# Autodesk Inventor assembly: Assembly1
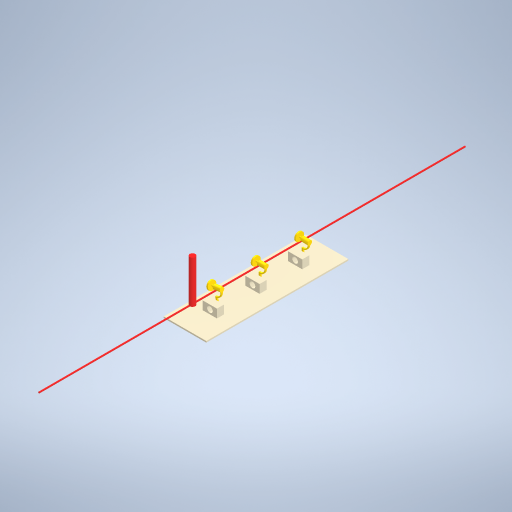
[picture p0: Inventor's stored thumbnail of the model, 512x512]
Saved by Autodesk Inventor 2024 (Build 280153000, 153)
## iProperties
Created: 2024-09-18
Part Number: Assembly1
Document SubType Name: Assembly
Designer: manas
Author: manas
## Documents named in this file (4)
- C:\Users\manas\Downloads\Assembly1.iam
- C:\Users\manas\Downloads\Part3.ipt
- C:\Users\manas\Downloads\Part2.ipt
- C:\Users\manas\Downloads\Part5.ipt
## Components (5 placed, 3 different names)
1. Part3:1 — Mate:1, Mate:2
2. Part2:1 — Mate:1, Mate:2, Mate:3, Mate:4, Mate:5, Mate:6
3. Part3:2 — Mate:3, Mate:4
4. Part3:3 — Mate:5, Mate:6
5. Part5:1
## Relationships (6: Mate 6)
- Mate:1: Part3:1 ↔ Part2:1
- Mate:2: Part3:1 ↔ Part2:1
- Mate:3: Part2:1 ↔ Part3:2
- Mate:4: Part2:1 ↔ Part3:2
- Mate:5: Part2:1 ↔ Part3:3
- Mate:6: Part2:1 ↔ Part3:3
